# Autodesk Inventor assembly: Top_Assy
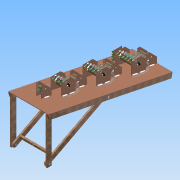
[picture p0: Inventor's stored thumbnail of the model, 180x180]
Saved by Autodesk Inventor 2018.1 (Build 221171000, 171)
## iProperties
Created: 2019-03-18
Part Number: Top_Assy
Document SubType Name: Assembly
Designer: James
Author: James
## Documents named in this file (19)
- C:\Users\admin\Desktop\Ball-Machine\Top Level\Top_Assy.iam
- C:\Users\admin\Desktop\Ball-Machine\Selection Sort\Selection_Assy.iam
- C:\Users\admin\Desktop\Ball-Machine\Pancake Sort\Pancake_Assy.iam
- C:\Users\admin\Desktop\Ball-Machine\Selection Sort\Selection - 4 Lanes\Selection_Assy 4 Lanes.iam
- C:\Users\admin\Desktop\Ball-Machine\Top Level\Top_Slider Assy.iam
- C:\Users\admin\Desktop\Ball-Machine\Selection Sort\Selection - 3 Lanes\Selection_Assy 3 Lanes.iam
- C:\Users\admin\Desktop\Ball-Machine\Selection Sort\Selection - 2 Lanes\Selection_Assy 2 Lanes.iam
- C:\Users\admin\Desktop\Ball-Machine\Pancake Sort\Pancake - 3 Lanes\Pancake_Assy_3 Lanes.iam
- C:\Users\admin\Desktop\Ball-Machine\Pancake Sort\Pancake - 4 Lanes\Pancake_Assy_4 Lanes.iam
- C:\Users\admin\Desktop\Ball-Machine\Top Level\Top_Slider Assy_3 Lanes.iam
- C:\Users\admin\Desktop\Ball-Machine\Top Level\Top_Slider Assy_4 Lanes.iam
- C:\Users\admin\Desktop\Ball-Machine\Top Level\Top_Backboard Assy.iam
- C:\Users\admin\Desktop\Ball-Machine\Top Level\Top_Angle Bracket Small.ipt
- C:\Users\admin\Desktop\Ball-Machine\Top Level\Nyloc Nut - M4.ipt
- C:\Users\admin\Desktop\Ball-Machine\Top Level\Socket Cap Screw - Standard - (A2) - M4 x 16.ipt
- C:\Users\admin\Desktop\Ball-Machine\Top Level\Socket Csk Screw - (A2) - M4 x  16.ipt
- C:\Users\admin\Desktop\Ball-Machine\Top Level\Pipes\Top_LHS Pipe.ipt
- C:\Users\admin\Desktop\Ball-Machine\Top Level\Pipes\Top_RHS Pipe.ipt
- C:\Users\admin\Desktop\Ball-Machine\Top Level\Top_Separator Assy.iam
## Components (60 placed, 18 different names)
1. Selection_Assy:1 [sub-assembly] — Flush:1, Flush:2, Flush:3, Flush:4, Flush:5, Mate:1, Tangent:1, Tangent:2, Mate:2, Flush:8, Flush:20, Mate:11, Mate:34, Mate:35, Mate:36, Mate:49, Mate:50, Mate:51
2. Pancake_Assy:1 [sub-assembly] — Flush:4, Mate:2, Flush:7, Mate:8, Mate:12
3. Selection_Assy 4 Lanes:1 [sub-assembly] — Flush:5, Flush:8, Flush:9, Mate:3, Flush:12, Mate:5, Mate:6, Tangent:3, Tangent:4, Flush:18, Mate:8, Mate:17, Mate:101, Mate:102, Mate:103, Mate:110, Mate:111, Mate:112
4. Top_Slider Assy:1 [sub-assembly] — Mate:1, Tangent:1, Tangent:2, Flush:7
5. Selection_Assy 3 Lanes:1 [sub-assembly] — Flush:9, Flush:10, Flush:13, Mate:4, Mate:7, Tangent:5, Tangent:6, Flush:19, Mate:9, Mate:15, Mate:104, Mate:105, Mate:106, Mate:107, Mate:108, Mate:109
6. Selection_Assy 2 Lanes:1 [sub-assembly] — Flush:10, Mate:10, Mate:13, Flush:21
7. Pancake_Assy_3 Lanes:1 [sub-assembly] — Flush:13, Mate:4, Mate:10, Mate:14
8. Pancake_Assy_4 Lanes:1 [sub-assembly] — Mate:3, Flush:12, Mate:9, Mate:16
9. Top_Slider Assy_3 Lanes:1 [sub-assembly] — Mate:7, Tangent:5, Tangent:6, Flush:19
10. Top_Slider Assy_4 Lanes:1 [sub-assembly] — Mate:5, Mate:6, Tangent:3, Tangent:4, Flush:18
11. Top_Backboard Assy:1 [sub-assembly] — Angle:1, Flush:20, Mate:11, Mate:12, Mate:13, Mate:14, Mate:15, Mate:16, Mate:17, Flush:21, Mate:113, Angle:8
12. Top_LHS Pipe:1 — Mate:37, Tangent:7, Angle:2
13. Top_RHS Pipe:1 — Tangent:8, Mate:52, Angle:3
14. Top_LHS Pipe:2
15. Top_RHS Pipe:2
16. Top_LHS Pipe:3
17. Top_RHS Pipe:3
18. Top_Separator Assy:1 [sub-assembly] — Mate:113, Angle:8
19. Top_Angle Bracket Small:3 — Mate:101
20. Nyloc Nut - M4:7
21. Socket Cap Screw - Standard - (A2) - M4 x 16:5 — Mate:103
22. Nyloc Nut - M4:8
23. Socket Csk Screw - (A2) - M4 x  16:3
24. Socket Cap Screw - Standard - (A2) - M4 x 16:6 — Mate:102
25. Nyloc Nut - M4:9
26. Top_Angle Bracket Small:4 — Mate:110
27. Nyloc Nut - M4:10
28. Socket Cap Screw - Standard - (A2) - M4 x 16:7 — Mate:112
29. Nyloc Nut - M4:11
30. Socket Csk Screw - (A2) - M4 x  16:4
31. Socket Cap Screw - Standard - (A2) - M4 x 16:8 — Mate:111
32. Nyloc Nut - M4:12
33. Top_Angle Bracket Small:5 — Mate:104
34. Nyloc Nut - M4:13
35. Socket Cap Screw - Standard - (A2) - M4 x 16:9 — Mate:106
36. Nyloc Nut - M4:14
37. Socket Csk Screw - (A2) - M4 x  16:5
38. Socket Cap Screw - Standard - (A2) - M4 x 16:10 — Mate:105
39. Nyloc Nut - M4:15
40. Top_Angle Bracket Small:6 — Mate:107
41. Nyloc Nut - M4:16
42. Socket Cap Screw - Standard - (A2) - M4 x 16:11 — Mate:109
43. Nyloc Nut - M4:17
44. Socket Csk Screw - (A2) - M4 x  16:6
45. Socket Cap Screw - Standard - (A2) - M4 x 16:12 — Mate:108
46. Nyloc Nut - M4:18
47. Top_Angle Bracket Small:2 — Mate:49, Tangent:8, Mate:52, Angle:3
48. Nyloc Nut - M4:4
49. Socket Cap Screw - Standard - (A2) - M4 x 16:3 — Mate:51
50. Nyloc Nut - M4:5
51. Socket Csk Screw - (A2) - M4 x  16:2
52. Socket Cap Screw - Standard - (A2) - M4 x 16:4 — Mate:50
53. Nyloc Nut - M4:6
54. Top_Angle Bracket Small:1 — Mate:18, Flush:22, Mate:21, Mate:28, Mate:29, Mate:32, Mate:33, Mate:36, Mate:37, Tangent:7, Angle:2
55. Nyloc Nut - M4:1 — Mate:21, Mate:22
56. Socket Cap Screw - Standard - (A2) - M4 x 16:1 — Mate:23, Mate:27, Mate:28, Mate:29, Mate:35
57. Nyloc Nut - M4:2 — Mate:23, Mate:27
58. Socket Csk Screw - (A2) - M4 x  16:1 — Mate:18, Flush:22, Mate:22
59. Socket Cap Screw - Standard - (A2) - M4 x 16:2 — Mate:32, Mate:33, Mate:34
60. Nyloc Nut - M4:3
## Relationships (149: Mate 108, Flush 21, Tangent 12, Angle 8)
- Flush:1: Selection_Assy:1
- Flush:2: Selection_Assy:1
- Flush:3: Selection_Assy:1
- Flush:4 (107.5 mm): Selection_Assy:1 ↔ Pancake_Assy:1
- Flush:5: Selection_Assy:1 ↔ Selection_Assy 4 Lanes:1
- Mate:1 (2 mm): Selection_Assy:1 ↔ Top_Slider Assy:1
- Tangent:1: Selection_Assy:1 ↔ Top_Slider Assy:1
- Tangent:2: Selection_Assy:1 ↔ Top_Slider Assy:1
- Mate:2 (160 mm): Selection_Assy:1 ↔ Pancake_Assy:1
- Flush:7: Pancake_Assy:1 ↔ Top_Slider Assy:1
- Flush:8: Selection_Assy:1 ↔ Selection_Assy 4 Lanes:1
- Flush:9: Selection_Assy 4 Lanes:1 ↔ Selection_Assy 3 Lanes:1
- Flush:10: Selection_Assy 3 Lanes:1 ↔ Selection_Assy 2 Lanes:1
- Mate:3 (160 mm): Selection_Assy 4 Lanes:1 ↔ Pancake_Assy_4 Lanes:1
- Flush:12 (62.5 mm): Selection_Assy 4 Lanes:1 ↔ Pancake_Assy_4 Lanes:1
- Flush:13 (17.5 mm): Selection_Assy 3 Lanes:1 ↔ Pancake_Assy_3 Lanes:1
- Mate:4 (160 mm): Selection_Assy 3 Lanes:1 ↔ Pancake_Assy_3 Lanes:1
- Mate:5 (2 mm): Selection_Assy 4 Lanes:1 ↔ Top_Slider Assy_4 Lanes:1
- Mate:6 (2 mm): Selection_Assy 4 Lanes:1 ↔ Top_Slider Assy_4 Lanes:1
- Tangent:3: Selection_Assy 4 Lanes:1 ↔ Top_Slider Assy_4 Lanes:1
- Tangent:4: Selection_Assy 4 Lanes:1 ↔ Top_Slider Assy_4 Lanes:1
- Flush:18: Selection_Assy 4 Lanes:1 ↔ Top_Slider Assy_4 Lanes:1
- Mate:7 (2 mm): Selection_Assy 3 Lanes:1 ↔ Top_Slider Assy_3 Lanes:1
- Tangent:5: Selection_Assy 3 Lanes:1 ↔ Top_Slider Assy_3 Lanes:1
- Tangent:6: Selection_Assy 3 Lanes:1 ↔ Top_Slider Assy_3 Lanes:1
- Flush:19: Selection_Assy 3 Lanes:1 ↔ Top_Slider Assy_3 Lanes:1
- Mate:8 (160 mm): Pancake_Assy:1 ↔ Selection_Assy 4 Lanes:1
- Mate:9 (160 mm): Selection_Assy 3 Lanes:1 ↔ Pancake_Assy_4 Lanes:1
- Mate:10 (160 mm): Selection_Assy 2 Lanes:1 ↔ Pancake_Assy_3 Lanes:1
- Angle:1 (0 deg): Top_Backboard Assy:1
- Flush:20 (-500 mm): Selection_Assy:1 ↔ Top_Backboard Assy:1
- Mate:11: Selection_Assy:1 ↔ Top_Backboard Assy:1
- Mate:12: Pancake_Assy:1 ↔ Top_Backboard Assy:1
- Mate:13: Selection_Assy 2 Lanes:1 ↔ Top_Backboard Assy:1
- Mate:14: Pancake_Assy_3 Lanes:1 ↔ Top_Backboard Assy:1
- Mate:15: Selection_Assy 3 Lanes:1 ↔ Top_Backboard Assy:1
- Mate:16: Pancake_Assy_4 Lanes:1 ↔ Top_Backboard Assy:1
- Mate:17: Selection_Assy 4 Lanes:1 ↔ Top_Backboard Assy:1
- Flush:21 (-400 mm): Selection_Assy 2 Lanes:1 ↔ Top_Backboard Assy:1
- Mate:18: Top_Angle Bracket Small:1 ↔ Socket Csk Screw - (A2) - M4 x  16:1
- Flush:22 (-5 mm): Top_Angle Bracket Small:1 ↔ Socket Csk Screw - (A2) - M4 x  16:1
- Mate:21: Top_Angle Bracket Small:1 ↔ Nyloc Nut - M4:1
- Mate:22: Nyloc Nut - M4:1 ↔ Socket Csk Screw - (A2) - M4 x  16:1
- Mate:23: Socket Cap Screw - Standard - (A2) - M4 x 16:1 ↔ Nyloc Nut - M4:2
- Mate:27 (8 mm): Socket Cap Screw - Standard - (A2) - M4 x 16:1 ↔ Nyloc Nut - M4:2
- Mate:28: Top_Angle Bracket Small:1 ↔ Socket Cap Screw - Standard - (A2) - M4 x 16:1
- Mate:29: Top_Angle Bracket Small:1 ↔ Socket Cap Screw - Standard - (A2) - M4 x 16:1
- [Mate]: Socket Cap Screw - Standard - (A2) - M4 x 16:2 ↔ Nyloc Nut - M4:3
- [Mate] (8 mm): Socket Cap Screw - Standard - (A2) - M4 x 16:2 ↔ Nyloc Nut - M4:3
- Mate:32: Top_Angle Bracket Small:1 ↔ Socket Cap Screw - Standard - (A2) - M4 x 16:2
- Mate:33: Top_Angle Bracket Small:1 ↔ Socket Cap Screw - Standard - (A2) - M4 x 16:2
- Mate:34: Selection_Assy:1 ↔ Socket Cap Screw - Standard - (A2) - M4 x 16:2
- Mate:35: Selection_Assy:1 ↔ Socket Cap Screw - Standard - (A2) - M4 x 16:1
- Mate:36: Selection_Assy:1 ↔ Top_Angle Bracket Small:1
- Mate:37: Top_LHS Pipe:1 ↔ Top_Angle Bracket Small:1
- Tangent:7: Top_LHS Pipe:1 ↔ Top_Angle Bracket Small:1
- Angle:2 (180 deg): Top_LHS Pipe:1 ↔ Top_Angle Bracket Small:1
- [Mate]: Top_Angle Bracket Small:2 ↔ Socket Csk Screw - (A2) - M4 x  16:2
- [Flush] (-5 mm): Top_Angle Bracket Small:2 ↔ Socket Csk Screw - (A2) - M4 x  16:2
- [Mate]: Top_Angle Bracket Small:2 ↔ Nyloc Nut - M4:4
- [Mate]: Nyloc Nut - M4:4 ↔ Socket Csk Screw - (A2) - M4 x  16:2
- [Mate]: Socket Cap Screw - Standard - (A2) - M4 x 16:3 ↔ Nyloc Nut - M4:5
- [Mate] (8 mm): Socket Cap Screw - Standard - (A2) - M4 x 16:3 ↔ Nyloc Nut - M4:5
- [Mate]: Top_Angle Bracket Small:2 ↔ Socket Cap Screw - Standard - (A2) - M4 x 16:3
- [Mate]: Top_Angle Bracket Small:2 ↔ Socket Cap Screw - Standard - (A2) - M4 x 16:3
- [Mate]: Socket Cap Screw - Standard - (A2) - M4 x 16:4 ↔ Nyloc Nut - M4:6
- [Mate] (8 mm): Socket Cap Screw - Standard - (A2) - M4 x 16:4 ↔ Nyloc Nut - M4:6
- [Mate]: Top_Angle Bracket Small:2 ↔ Socket Cap Screw - Standard - (A2) - M4 x 16:4
- [Mate]: Top_Angle Bracket Small:2 ↔ Socket Cap Screw - Standard - (A2) - M4 x 16:4
- Mate:49: Selection_Assy:1 ↔ Top_Angle Bracket Small:2
- Mate:50: Selection_Assy:1 ↔ Socket Cap Screw - Standard - (A2) - M4 x 16:4
- Mate:51: Selection_Assy:1 ↔ Socket Cap Screw - Standard - (A2) - M4 x 16:3
- Tangent:8: Top_RHS Pipe:1 ↔ Top_Angle Bracket Small:2
- Mate:52: Top_RHS Pipe:1 ↔ Top_Angle Bracket Small:2
- Angle:3 (180 deg): Top_RHS Pipe:1 ↔ Top_Angle Bracket Small:2
- [Mate]: Top_Angle Bracket Small:3 ↔ Socket Csk Screw - (A2) - M4 x  16:3
- [Flush] (-5 mm): Top_Angle Bracket Small:3 ↔ Socket Csk Screw - (A2) - M4 x  16:3
- [Mate]: Top_Angle Bracket Small:3 ↔ Nyloc Nut - M4:7
- [Mate]: Nyloc Nut - M4:7 ↔ Socket Csk Screw - (A2) - M4 x  16:3
- [Mate]: Socket Cap Screw - Standard - (A2) - M4 x 16:5 ↔ Nyloc Nut - M4:8
- [Mate] (8 mm): Socket Cap Screw - Standard - (A2) - M4 x 16:5 ↔ Nyloc Nut - M4:8
- [Mate]: Top_Angle Bracket Small:3 ↔ Socket Cap Screw - Standard - (A2) - M4 x 16:5
- [Mate]: Top_Angle Bracket Small:3 ↔ Socket Cap Screw - Standard - (A2) - M4 x 16:5
- [Mate]: Socket Cap Screw - Standard - (A2) - M4 x 16:6 ↔ Nyloc Nut - M4:9
- [Mate] (8 mm): Socket Cap Screw - Standard - (A2) - M4 x 16:6 ↔ Nyloc Nut - M4:9
- [Mate]: Top_Angle Bracket Small:3 ↔ Socket Cap Screw - Standard - (A2) - M4 x 16:6
- [Mate]: Top_Angle Bracket Small:3 ↔ Socket Cap Screw - Standard - (A2) - M4 x 16:6
- [Mate]: Top_LHS Pipe:2 ↔ Top_Angle Bracket Small:3
- [Tangent]: Top_LHS Pipe:2 ↔ Top_Angle Bracket Small:3
- [Angle] (180 deg): Top_LHS Pipe:2 ↔ Top_Angle Bracket Small:3
- [Mate]: Top_Angle Bracket Small:4 ↔ Socket Csk Screw - (A2) - M4 x  16:4
- [Flush] (-5 mm): Top_Angle Bracket Small:4 ↔ Socket Csk Screw - (A2) - M4 x  16:4
- [Mate]: Top_Angle Bracket Small:4 ↔ Nyloc Nut - M4:10
- [Mate]: Nyloc Nut - M4:10 ↔ Socket Csk Screw - (A2) - M4 x  16:4
- [Mate]: Socket Cap Screw - Standard - (A2) - M4 x 16:7 ↔ Nyloc Nut - M4:11
- [Mate] (8 mm): Socket Cap Screw - Standard - (A2) - M4 x 16:7 ↔ Nyloc Nut - M4:11
- [Mate]: Top_Angle Bracket Small:4 ↔ Socket Cap Screw - Standard - (A2) - M4 x 16:7
- [Mate]: Top_Angle Bracket Small:4 ↔ Socket Cap Screw - Standard - (A2) - M4 x 16:7
- [Mate]: Socket Cap Screw - Standard - (A2) - M4 x 16:8 ↔ Nyloc Nut - M4:12
- [Mate] (8 mm): Socket Cap Screw - Standard - (A2) - M4 x 16:8 ↔ Nyloc Nut - M4:12
- [Mate]: Top_Angle Bracket Small:4 ↔ Socket Cap Screw - Standard - (A2) - M4 x 16:8
- [Mate]: Top_Angle Bracket Small:4 ↔ Socket Cap Screw - Standard - (A2) - M4 x 16:8
- [Tangent]: Top_RHS Pipe:2 ↔ Top_Angle Bracket Small:4
- [Mate]: Top_RHS Pipe:2 ↔ Top_Angle Bracket Small:4
- [Angle] (180 deg): Top_RHS Pipe:2 ↔ Top_Angle Bracket Small:4
- [Mate]: Top_Angle Bracket Small:5 ↔ Socket Csk Screw - (A2) - M4 x  16:5
- [Flush] (-5 mm): Top_Angle Bracket Small:5 ↔ Socket Csk Screw - (A2) - M4 x  16:5
- [Mate]: Top_Angle Bracket Small:5 ↔ Nyloc Nut - M4:13
- [Mate]: Nyloc Nut - M4:13 ↔ Socket Csk Screw - (A2) - M4 x  16:5
- [Mate]: Socket Cap Screw - Standard - (A2) - M4 x 16:9 ↔ Nyloc Nut - M4:14
- [Mate] (8 mm): Socket Cap Screw - Standard - (A2) - M4 x 16:9 ↔ Nyloc Nut - M4:14
- [Mate]: Top_Angle Bracket Small:5 ↔ Socket Cap Screw - Standard - (A2) - M4 x 16:9
- [Mate]: Top_Angle Bracket Small:5 ↔ Socket Cap Screw - Standard - (A2) - M4 x 16:9
- [Mate]: Socket Cap Screw - Standard - (A2) - M4 x 16:10 ↔ Nyloc Nut - M4:15
- [Mate] (8 mm): Socket Cap Screw - Standard - (A2) - M4 x 16:10 ↔ Nyloc Nut - M4:15
- [Mate]: Top_Angle Bracket Small:5 ↔ Socket Cap Screw - Standard - (A2) - M4 x 16:10
- [Mate]: Top_Angle Bracket Small:5 ↔ Socket Cap Screw - Standard - (A2) - M4 x 16:10
- [Mate]: Top_LHS Pipe:3 ↔ Top_Angle Bracket Small:5
- [Tangent]: Top_LHS Pipe:3 ↔ Top_Angle Bracket Small:5
- [Angle] (180 deg): Top_LHS Pipe:3 ↔ Top_Angle Bracket Small:5
- [Mate]: Top_Angle Bracket Small:6 ↔ Socket Csk Screw - (A2) - M4 x  16:6
- [Flush] (-5 mm): Top_Angle Bracket Small:6 ↔ Socket Csk Screw - (A2) - M4 x  16:6
- [Mate]: Top_Angle Bracket Small:6 ↔ Nyloc Nut - M4:16
- [Mate]: Nyloc Nut - M4:16 ↔ Socket Csk Screw - (A2) - M4 x  16:6
- [Mate]: Socket Cap Screw - Standard - (A2) - M4 x 16:11 ↔ Nyloc Nut - M4:17
- [Mate] (8 mm): Socket Cap Screw - Standard - (A2) - M4 x 16:11 ↔ Nyloc Nut - M4:17
- [Mate]: Top_Angle Bracket Small:6 ↔ Socket Cap Screw - Standard - (A2) - M4 x 16:11
- [Mate]: Top_Angle Bracket Small:6 ↔ Socket Cap Screw - Standard - (A2) - M4 x 16:11
- [Mate]: Socket Cap Screw - Standard - (A2) - M4 x 16:12 ↔ Nyloc Nut - M4:18
- [Mate] (8 mm): Socket Cap Screw - Standard - (A2) - M4 x 16:12 ↔ Nyloc Nut - M4:18
- [Mate]: Top_Angle Bracket Small:6 ↔ Socket Cap Screw - Standard - (A2) - M4 x 16:12
- [Mate]: Top_Angle Bracket Small:6 ↔ Socket Cap Screw - Standard - (A2) - M4 x 16:12
- [Tangent]: Top_RHS Pipe:3 ↔ Top_Angle Bracket Small:6
- [Mate]: Top_RHS Pipe:3 ↔ Top_Angle Bracket Small:6
- [Angle] (180 deg): Top_RHS Pipe:3 ↔ Top_Angle Bracket Small:6
- Mate:101: Selection_Assy 4 Lanes:1 ↔ Top_Angle Bracket Small:3
- Mate:102: Selection_Assy 4 Lanes:1 ↔ Socket Cap Screw - Standard - (A2) - M4 x 16:6
- Mate:103: Selection_Assy 4 Lanes:1 ↔ Socket Cap Screw - Standard - (A2) - M4 x 16:5
- Mate:104: Selection_Assy 3 Lanes:1 ↔ Top_Angle Bracket Small:5
- Mate:105: Selection_Assy 3 Lanes:1 ↔ Socket Cap Screw - Standard - (A2) - M4 x 16:10
- Mate:106: Selection_Assy 3 Lanes:1 ↔ Socket Cap Screw - Standard - (A2) - M4 x 16:9
- Mate:107: Selection_Assy 3 Lanes:1 ↔ Top_Angle Bracket Small:6
- Mate:108: Selection_Assy 3 Lanes:1 ↔ Socket Cap Screw - Standard - (A2) - M4 x 16:12
- Mate:109: Selection_Assy 3 Lanes:1 ↔ Socket Cap Screw - Standard - (A2) - M4 x 16:11
- Mate:110: Selection_Assy 4 Lanes:1 ↔ Top_Angle Bracket Small:4
- Mate:111: Selection_Assy 4 Lanes:1 ↔ Socket Cap Screw - Standard - (A2) - M4 x 16:8
- Mate:112: Selection_Assy 4 Lanes:1 ↔ Socket Cap Screw - Standard - (A2) - M4 x 16:7
- Mate:113: Top_Backboard Assy:1 ↔ Top_Separator Assy:1
- Angle:8 (0 deg): Top_Backboard Assy:1 ↔ Top_Separator Assy:1
## Named parameters: d87_d79 = 0 mm, d88_d84 = 8 mm, d97_d73 = 0 mm, d98_d85 = 0 mm, d99_d86 = 0 mm, d100_d87_d79 = 0 mm, d101_d88_d84 = 8 mm, d102_d89 = 0 mm, d103_d90 = 0 mm, d104_d74 = -5 mm, d105_d77 = 0 mm, d106_d78 = 0 mm, d107_d79 = 0 mm, d108_d84 = 8 mm, d115_d73 = 0 mm, d116_d104_d74 = -5 mm, d117_d105_d77 = 0 mm, d118_d106_d78 = 0 mm, d119_d107_d79 = 0 mm, d120_d108_d84 = 8 mm, d121_d112 = 0 mm, d122_d113 = 0 mm, d123_d114 = 180 deg, d124_d85 = 0 mm, d125_d86 = 0 mm, d126_d87_d79 = 0 mm, d127_d88_d84 = 8 mm, d128_d89 = 0 mm, d129_d90 = 0 mm, d130_d94 = 0 mm, d131_d95 = 0 mm, d132_d96 = 180 deg, d133_d97_d73 = 0 mm, d134_d98_d85 = 0 mm, d135_d99_d86 = 0 mm, d136_d100_d87_d79 = 0 mm, d137_d101_d88_d84 = 8 mm, d138_d102_d89 = 0 mm, d139_d103_d90 = 0 mm, d140_d74 = -5 mm, d141_d77 = 0 mm, d142_d78 = 0 mm, d143_d79 = 0 mm, d144_d84 = 8 mm, d145_d73 = 0 mm, d146_d104_d74 = -5 mm, d147_d105_d77 = 0 mm, d148_d106_d78 = 0 mm, d149_d107_d79 = 0 mm, d150_d108_d84 = 8 mm, d151_d112 = 0 mm, d152_d113 = 0 mm, d153_d114 = 180 deg, d154_d85 = 0 mm, d155_d86 = 0 mm, d156_d87_d79 = 0 mm, d157_d88_d84 = 8 mm, d158_d89 = 0 mm, d159_d90 = 0 mm, d160_d94 = 0 mm, d161_d95 = 0 mm, d162_d96 = 180 deg, d163_d97_d73 = 0 mm, d164_d98_d85 = 0 mm, d165_d99_d86 = 0 mm, d166_d100_d87_d79 = 0 mm, d167_d101_d88_d84 = 8 mm, d168_d102_d89 = 0 mm, d169_d103_d90 = 0 mm, d170_d74 = -5 mm, d171_d77 = 0 mm, d172_d78 = 0 mm, d173_d79 = 0 mm, d174_d84 = 8 mm
